# Autodesk Inventor assembly: torso_link
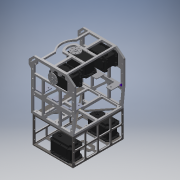
[picture p0: Inventor's stored thumbnail of the model, 180x180]
Saved by Autodesk Inventor 2018 (Build 220112000, 112)
## iProperties
Created: 2018-11-26
Part Number: torso_link
Document SubType Name: Assembly
Designer: bitbots
Mass: 613.238 g
Surface Area: 2643.37 cm^2
Volume: 613.238 cm^3
Density: 1 g/cm^3
Author: bitbots
## Documents named in this file (9)
- C:\Users\jaspe\bitbots_hardware\wolfgang\assembly\body\torso_link.iam
- C:\Users\jaspe\bitbots_hardware\wolfgang\assembly\body\torso_bottom.ipt
- C:\Users\jaspe\bitbots_hardware\wolfgang\assembly\body\torso_top.ipt
- C:\Users\jaspe\bitbots_hardware\wolfgang\assembly\motors\MX64\Mx64_with_horn.iam
- C:\Users\jaspe\bitbots_hardware\wolfgang\assembly\motors\MX106\MX-106_with_horn.iam
- C:\Users\jaspe\bitbots_hardware\Nimbro_Teile\Nimbro-OP-Master-CAD\IGS 3D\right_hip_yaw_link.ipt
- C:\Users\jaspe\bitbots_hardware\wolfgang\assembly\body\hip_z_spacer.ipt
- C:\Users\jaspe\bitbots_hardware\wolfgang\assembly\body\nuc_holdingrail_left.ipt
- C:\Users\jaspe\bitbots_hardware\wolfgang\assembly\body\nuc_holdingrail_right.ipt
## Components (14 placed, 8 different names)
1. torso_bottom:1 — Mate:14, Mate:15, Mate:16, Mate:26, Mate:27, Mate:29, Mate:30, Mate:39, Mate:40, Mate:41, Mate:42, Mate:43, Flush:35, Mate:44, Mate:45, Mate:46, Mate:47, Mate:48, Flush:36
2. torso_top:1 — Mate:14, Mate:15, Mate:16, Mate:17, Mate:18, Mate:19, Mate:20, Mate:21, Mate:22, Mate:23, Mate:24, Mate:25, Flush:34, Mate:34, Angle:1, Mate:35, Angle:2, Mate:49, Mate:50, Mate:51, Mate:52, Mate:53, Mate:54
3. Mx64_with_horn:1 [sub-assembly] — Mate:23, Mate:24, Mate:25
4. Mx64_with_horn:2 [sub-assembly] — Mate:17, Mate:18, Mate:19
5. Mx64_with_horn:3 [sub-assembly] — Mate:20, Mate:21, Mate:22
6. MX-106_with_horn:1 [sub-assembly] — Mate:26, Mate:27
7. MX-106_with_horn:2 [sub-assembly] — Mate:29, Mate:30, Flush:37, Mate:55
8. right_hip_yaw_link:1
9. hip_z_spacer:1 — Mate:39, Mate:40, Mate:41
10. hip_z_spacer:2 — Mate:42, Mate:43, Flush:35
11. hip_z_spacer:3 — Mate:47, Mate:48, Flush:36
12. hip_z_spacer:4 — Mate:44, Mate:45, Mate:46, Flush:37
13. nuc_holdingrail_left:1 — Mate:49, Mate:50, Mate:51
14. nuc_holdingrail_right:1 — Mate:52, Mate:53, Mate:54
## Relationships (44: Mate 37, Flush 4, Angle 2, Symmetry 1)
- Mate:14: torso_bottom:1 ↔ torso_top:1
- Mate:15: torso_bottom:1 ↔ torso_top:1
- Mate:16: torso_bottom:1 ↔ torso_top:1
- Mate:17: torso_top:1 ↔ Mx64_with_horn:2
- Mate:18: torso_top:1 ↔ Mx64_with_horn:2
- Mate:19: torso_top:1 ↔ Mx64_with_horn:2
- Mate:20: torso_top:1 ↔ Mx64_with_horn:3
- Mate:21: torso_top:1 ↔ Mx64_with_horn:3
- Mate:22: torso_top:1 ↔ Mx64_with_horn:3
- Mate:23: torso_top:1 ↔ Mx64_with_horn:1
- Mate:24: torso_top:1 ↔ Mx64_with_horn:1
- Mate:25: torso_top:1 ↔ Mx64_with_horn:1
- Mate:26: torso_bottom:1 ↔ MX-106_with_horn:1
- Mate:27: torso_bottom:1 ↔ MX-106_with_horn:1
- Mate:29: torso_bottom:1 ↔ MX-106_with_horn:2
- Mate:30: torso_bottom:1 ↔ MX-106_with_horn:2
- Flush:34: torso_top:1
- Mate:34: torso_top:1
- Angle:1 (0 deg): torso_top:1
- Mate:35: torso_top:1
- Angle:2 (0 deg): torso_top:1
- Symmetry:1
- Mate:37
- Mate:38
- Mate:39: torso_bottom:1 ↔ hip_z_spacer:1
- Mate:40: torso_bottom:1 ↔ hip_z_spacer:1
- Mate:41: torso_bottom:1 ↔ hip_z_spacer:1
- Mate:42: torso_bottom:1 ↔ hip_z_spacer:2
- Mate:43: torso_bottom:1 ↔ hip_z_spacer:2
- Flush:35: torso_bottom:1 ↔ hip_z_spacer:2
- Mate:44: torso_bottom:1 ↔ hip_z_spacer:4
- Mate:45: torso_bottom:1 ↔ hip_z_spacer:4
- Mate:46: torso_bottom:1 ↔ hip_z_spacer:4
- Mate:47: torso_bottom:1 ↔ hip_z_spacer:3
- Mate:48: torso_bottom:1 ↔ hip_z_spacer:3
- Flush:36: torso_bottom:1 ↔ hip_z_spacer:3
- Flush:37: MX-106_with_horn:2 ↔ hip_z_spacer:4
- Mate:49: torso_top:1 ↔ nuc_holdingrail_left:1
- Mate:50: torso_top:1 ↔ nuc_holdingrail_left:1
- Mate:51: torso_top:1 ↔ nuc_holdingrail_left:1
- Mate:52: torso_top:1 ↔ nuc_holdingrail_right:1
- Mate:53: torso_top:1 ↔ nuc_holdingrail_right:1
- Mate:54: torso_top:1 ↔ nuc_holdingrail_right:1
- Mate:55 (55 mm): MX-106_with_horn:2
